# Autodesk Inventor assembly: E-Axis v2.0
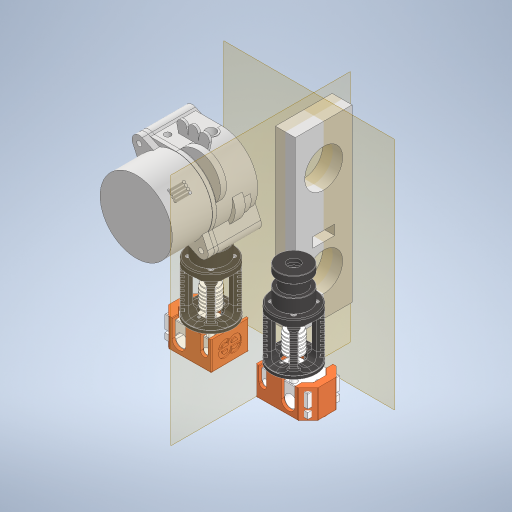
[picture p0: Inventor's stored thumbnail of the model, 512x512]
Saved by Autodesk Inventor 2023 (Build 270158000, 158)
## iProperties
Created: 2023-07-26
Part Number: E-Axis v2.0
Document SubType Name: Assembly
Designer: Parker
Author: Parker
## Documents named in this file (4)
- D:\000 - PEPCORP CLOUD\00- Legacy\Designs\MK3PRO P1\E-Axis\E-Axis v2.0.iam
- D:\000 - PEPCORP CLOUD\00- Legacy\Designs\MK3PRO P1\E-Axis\Solid1.ipt
- D:\000 - PEPCORP CLOUD\00- Legacy\Designs\MK3PRO P1\E-Axis\LGX-Lite-Simplified-V6.step\LGX-Lite-Simplified-V6.ipt
- D:\000 - PEPCORP CLOUD\00- Legacy\Designs\MK3PRO P1\E-Axis\Dragon hotend.iam
## Components (4 placed, 3 different names)
1. Solid1:1 — Mate:2
2. LGX-Lite-Simplified-V6:1 — Mate:2, Mate:3, Mate:4, Mate:5
3. Dragon hotend:1 [sub-assembly] — Mate:3, Mate:4, Flush:1, Angle:1, Mate:8
4. Dragon hotend:2 [sub-assembly] — Flush:1, Angle:1, Mate:6, Mate:7
## Relationships (9: Mate 7, Flush 1, Angle 1)
- Mate:2 (-40 mm): Solid1:1 ↔ LGX-Lite-Simplified-V6:1
- Mate:3: LGX-Lite-Simplified-V6:1 ↔ Dragon hotend:1
- Mate:4: LGX-Lite-Simplified-V6:1 ↔ Dragon hotend:1
- Mate:5 (-6 mm): LGX-Lite-Simplified-V6:1
- Flush:1 (1 mm): Dragon hotend:1 ↔ Dragon hotend:2
- Angle:1 (180 deg): Dragon hotend:1 ↔ Dragon hotend:2
- Mate:6 (20 mm): Dragon hotend:2
- Mate:7 (30 mm): Dragon hotend:2
- Mate:8 (30 mm): Dragon hotend:1
